# Autodesk Inventor assembly: Mark 6
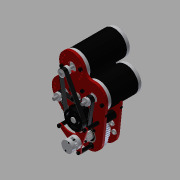
[picture p0: Inventor's stored thumbnail of the model, 180x180]
Saved by Autodesk Inventor 2013 (Build 170138000, 138)
## iProperties
Created: 2013-10-31
Part Number: Mark 6
Document SubType Name: Assembly
Designer: grtstudent
Author: grtstudent
## Documents named in this file (9)
- C:\Users\grtstudent\Desktop\Mark 6 Final Preseason\Mark 6.iam
- C:\Users\grtstudent\Desktop\Mark 6 Final Preseason\Mark 6 - Frame.iam
- C:\Users\grtstudent\Desktop\Mark 6 Final Preseason\Mark 6 - Cluster Shaft.iam
- C:\Users\grtstudent\Desktop\Mark 6 Final Preseason\Mark 6 - Output Shaft.iam
- C:\Users\grtstudent\Desktop\Mark 6 Final Preseason\Mark 6 - Pnuematic Assembly.iam
- C:\Users\grtstudent\Desktop\Mark 6 Final Preseason\Belts\267 mm Belt.ipt
- C:\Users\grtstudent\Desktop\Mark 6 Final Preseason\Belts\285 mm Belt.ipt
- C:\Users\grtstudent\Desktop\Mark 6 Final Preseason\Pulleys\16T 3mm GT2 - 8mm Key Broach.ipt
- C:\Users\grtstudent\Desktop\Mark 6 Final Preseason\Encoder\S4-120-250-N-S-B.ipt
## Components (10 placed, 8 different names)
1. Mark 6 - Frame:1 [sub-assembly] — Mate:1, Mate:2, Mate:4, Flush:1, Mate:5, Mate:6, Mate:9, Mate:11, Mate:12, Mate:15, Mate:16, Mate:17, Mate:19, Mate:20, Flush:4, Flush:5, Flush:6
2. Mark 6 - Cluster Shaft:1 [sub-assembly] — Mate:1, Mate:2, Mate:8, Mate:10, Mate:13, Mate:14
3. Mark 6 - Output Shaft:1 [sub-assembly] — Mate:3, Mate:4, Flush:1
4. Mark 6 - Pnuematic Assembly:1 [sub-assembly] — Mate:3, Mate:5, Mate:6
5. S4-120-250-N-S-B:1 — Mate:19, Mate:20
6. 285 mm Belt:1 — Mate:8, Mate:9, Mate:14, Mate:18
7. 267 mm Belt:1 — Mate:10, Mate:11, Mate:12, Mate:13, Flush:2, Flush:3
8. 16T 3mm GT2 - 8mm Key Broach:1 — Mate:17, Flush:2, Flush:6
9. 16T 3mm GT2 - 8mm Key Broach:2 — Mate:15, Flush:3, Flush:5
10. 16T 3mm GT2 - 8mm Key Broach:3 — Mate:16, Mate:18, Flush:4
## Relationships (25: Mate 19, Flush 6)
- Mate:1: Mark 6 - Frame:1 ↔ Mark 6 - Cluster Shaft:1
- Mate:2: Mark 6 - Frame:1 ↔ Mark 6 - Cluster Shaft:1
- Mate:3: Mark 6 - Output Shaft:1 ↔ Mark 6 - Pnuematic Assembly:1
- Mate:4: Mark 6 - Frame:1 ↔ Mark 6 - Output Shaft:1
- Flush:1: Mark 6 - Frame:1 ↔ Mark 6 - Output Shaft:1
- Mate:5: Mark 6 - Frame:1 ↔ Mark 6 - Pnuematic Assembly:1
- Mate:6: Mark 6 - Frame:1 ↔ Mark 6 - Pnuematic Assembly:1
- Mate:8: Mark 6 - Cluster Shaft:1 ↔ 285 mm Belt:1
- Mate:9: Mark 6 - Frame:1 ↔ 285 mm Belt:1
- Mate:10: Mark 6 - Cluster Shaft:1 ↔ 267 mm Belt:1
- Mate:11: Mark 6 - Frame:1 ↔ 267 mm Belt:1
- Mate:12: Mark 6 - Frame:1 ↔ 267 mm Belt:1
- Mate:13: Mark 6 - Cluster Shaft:1 ↔ 267 mm Belt:1
- Mate:14: Mark 6 - Cluster Shaft:1 ↔ 285 mm Belt:1
- Mate:15: Mark 6 - Frame:1 ↔ 16T 3mm GT2 - 8mm Key Broach:2
- Mate:16: Mark 6 - Frame:1 ↔ 16T 3mm GT2 - 8mm Key Broach:3
- Mate:17: Mark 6 - Frame:1 ↔ 16T 3mm GT2 - 8mm Key Broach:1
- Mate:18: 285 mm Belt:1 ↔ 16T 3mm GT2 - 8mm Key Broach:3
- Flush:2: 267 mm Belt:1 ↔ 16T 3mm GT2 - 8mm Key Broach:1
- Flush:3: 267 mm Belt:1 ↔ 16T 3mm GT2 - 8mm Key Broach:2
- Mate:19: Mark 6 - Frame:1 ↔ S4-120-250-N-S-B:1
- Mate:20: Mark 6 - Frame:1 ↔ S4-120-250-N-S-B:1
- Flush:4: Mark 6 - Frame:1 ↔ 16T 3mm GT2 - 8mm Key Broach:3
- Flush:5: Mark 6 - Frame:1 ↔ 16T 3mm GT2 - 8mm Key Broach:2
- Flush:6: Mark 6 - Frame:1 ↔ 16T 3mm GT2 - 8mm Key Broach:1
